# Autodesk Inventor assembly: Front A Assembly
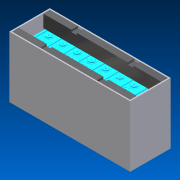
[picture p0: Inventor's stored thumbnail of the model, 180x180]
Saved by Autodesk Inventor 2012 (Build 160160000, 160)
## iProperties
Created: 2012-07-01
Part Number: Front A Assembly
Document SubType Name: Assembly
Designer: Hemant
Author: Hemant
## Documents named in this file (4)
- C:\Users\Hemant\Documents\Battery Boxes\BB FRONT A\Front A Assembly.iam
- C:\Users\Hemant\Documents\Battery Boxes\BB FRONT A\Small Battery Box Pastic 1.ipt
- C:\Users\Hemant\Documents\Battery Boxes\Batteries\Front A Battery Pack.iam
- C:\Users\Hemant\Documents\Battery Boxes\BB FRONT A\BB FRONT A SPACER 1.ipt
## Components (4 placed, 3 different names)
1. Small Battery Box Pastic 1:1 — Mate:1, Mate:2, Mate:3, Mate:5, Mate:6
2. Front A Battery Pack:1 [sub-assembly] — Mate:1, Mate:2, Mate:3, Mate:4
3. BB FRONT A SPACER 1:1 — Mate:4, Mate:5, Mate:6
4. BB FRONT A SPACER 1:2
## Component patterns: (2 elements, first: BB FRONT A SPACER 1:1)
## Relationships (6: Mate 6)
- Mate:1: Small Battery Box Pastic 1:1 ↔ Front A Battery Pack:1
- Mate:2 (8.4074 mm): Small Battery Box Pastic 1:1 ↔ Front A Battery Pack:1
- Mate:3 (16.3068 mm): Small Battery Box Pastic 1:1 ↔ Front A Battery Pack:1
- Mate:4: Front A Battery Pack:1 ↔ BB FRONT A SPACER 1:1
- Mate:5: Small Battery Box Pastic 1:1 ↔ BB FRONT A SPACER 1:1
- Mate:6: Small Battery Box Pastic 1:1 ↔ BB FRONT A SPACER 1:1
